# Autodesk Inventor assembly: quase tudo pronto
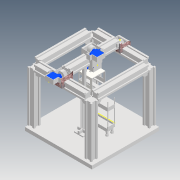
[picture p0: Inventor's stored thumbnail of the model, 180x180]
Saved by Autodesk Inventor 2021 (Build 250183000, 183)
## iProperties
Created: 2020-10-09
Part Number: quase tudo pronto
Document SubType Name: Assembly
Designer: evert
Author: evert
## Documents named in this file (16)
- C:\Users\evert\OneDrive\Área de Trabalho\peca move\quase tudo pronto.iam
- C:\Users\evert\OneDrive\Área de Trabalho\peca move\Peça16.ipt
- C:\Users\evert\OneDrive\Área de Trabalho\peca move\Viga_Projeto_Bosch.ipt
- C:\Users\evert\OneDrive\Área de Trabalho\peca move\elevador_caixa_com_estabi_v2 (2).ipt
- C:\Users\evert\OneDrive\Área de Trabalho\peca move\Viga_Projeto_Bosch (1).ipt
- C:\Users\evert\OneDrive\Área de Trabalho\peca move\Peça1,61.ipt
- C:\Users\evert\OneDrive\Área de Trabalho\peca move\sup movi.ipt
- C:\Users\evert\OneDrive\Área de Trabalho\peca move\roda sup.ipt
- C:\Users\evert\OneDrive\Área de Trabalho\peca move\viga de suporte.ipt
- C:\Users\evert\OneDrive\Área de Trabalho\peca move\Servo Motor SG90.ipt
- C:\Users\evert\OneDrive\Área de Trabalho\peca move\roda certa.ipt
- C:\Users\evert\OneDrive\Área de Trabalho\peca move\roda certa 2.0.ipt
- C:\Users\evert\OneDrive\Área de Trabalho\peca move\roda corda.ipt
- C:\Users\evert\OneDrive\Área de Trabalho\peca move\aramzem diferenciado beta 2.ipt
- C:\Users\evert\OneDrive\Área de Trabalho\peca move\base.ipt
- C:\Users\evert\OneDrive\Área de Trabalho\peca move\stl\suporte para arma.ipt
## Components (23 placed, 15 different names)
1. Peça16:1 — Conjunto de gaveta:1, Rígida:1, Rígida:5, Rotativa:12, Rígida:8
2. Viga_Projeto_Bosch:1 — Conjunto de gaveta:1
3. elevador_caixa_com_estabi_v2 (2):1 — Rígida:1
4. Viga_Projeto_Bosch (1):1 — Rígida:3
5. Viga_Projeto_Bosch (1):2 — Rígida:4
6. Viga_Projeto_Bosch (1):3
7. Viga_Projeto_Bosch (1):4
8. Peça1,61:1 — Rígida:3, Rotativa:13, Rígida:9
9. sup movi:1 — Rígida:4, Rotativa:7
10. roda sup:1 — Rotativa:7
11. viga de suporte:1
12. viga de suporte:2
13. viga de suporte:3
14. viga de suporte:4 — Rígida:10
15. Servo Motor SG90:1 — Rígida:5, Rotativa:14
16. roda certa:1 — Rotativa:12
17. Servo Motor SG90:4 — Rígida:8
18. roda certa 2.0:1 — Rotativa:13
19. Servo Motor SG90:5 — Rígida:9
20. roda corda:1 — Rotativa:14
21. aramzem diferenciado beta 2:1 — Rígida:11
22. base:1 — Rígida:10, Rígida:11
23. suporte para arma:1
## Relationships (13: WeldJoint 8, RevoluteJoint 4, TranslationJoint 1)
- Conjunto de gaveta:1 [TranslationJoint]: Peça16:1 ↔ Viga_Projeto_Bosch:1
- Rígida:1 [WeldJoint]: Peça16:1 ↔ elevador_caixa_com_estabi_v2 (2):1
- Rígida:3 [WeldJoint]: Viga_Projeto_Bosch (1):1 ↔ Peça1,61:1
- Rígida:4 [WeldJoint]: Viga_Projeto_Bosch (1):2 ↔ sup movi:1
- Rotativa:7 [RevoluteJoint]: sup movi:1 ↔ roda sup:1
- Rígida:5 [WeldJoint]: Peça16:1 ↔ Servo Motor SG90:1
- Rotativa:12 [RevoluteJoint]: Peça16:1 ↔ roda certa:1
- Rígida:8 [WeldJoint]: Peça16:1 ↔ Servo Motor SG90:4
- Rotativa:13 [RevoluteJoint]: Peça1,61:1 ↔ roda certa 2.0:1
- Rígida:9 [WeldJoint]: Peça1,61:1 ↔ Servo Motor SG90:5
- Rotativa:14 [RevoluteJoint]: Servo Motor SG90:1 ↔ roda corda:1
- Rígida:10 [WeldJoint]: viga de suporte:4 ↔ base:1
- Rígida:11 [WeldJoint]: aramzem diferenciado beta 2:1 ↔ base:1
